# Autodesk Inventor assembly: New_Tail
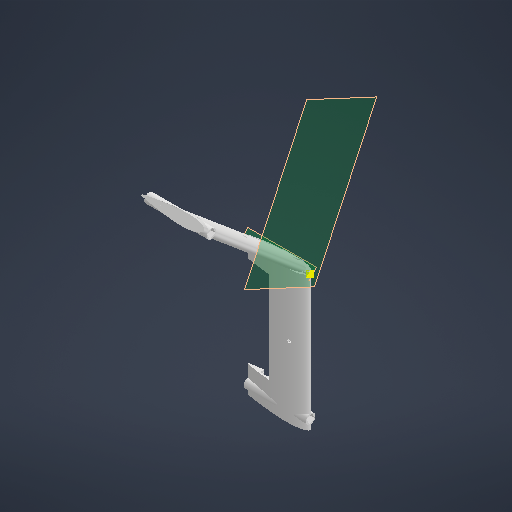
[picture p0: Inventor's stored thumbnail of the model, 512x512]
Saved by Autodesk Inventor 2026 (Build 300175050, 175E)
## iProperties
Created: 2026-06-16
Part Number: New_Tail
Document SubType Name: Assembly
Designer: Delbe
Author: Delbe
## Documents named in this file (3)
- C:\GitHub\SWIFT-UAV\System_development\Pelican\structural_model\v0.3.0\Parts\Delb_Parts\New_Tail.iam
- C:\GitHub\SWIFT-UAV\System_development\Pelican\structural_model\v0.3.0\Parts\Delb_Parts\Delb_Tail_Female_v1.ipt
- C:\GitHub\SWIFT-UAV\System_development\Pelican\structural_model\v0.3.0\Parts\Delb_Parts\Delb_Tail_Mirror_yea.ipt
## Components (2 placed, 2 different names)
1. Delb_Tail_Female_v1:1 — Mate:1
2. Delb_Tail_Mirror_yea:1 — Mate:1
## Relationships (1: Mate 1)
- Mate:1: Delb_Tail_Female_v1:1 ↔ Delb_Tail_Mirror_yea:1
